# Autodesk Inventor assembly: forklift_1_0
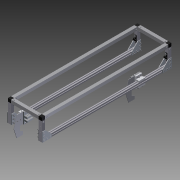
[picture p0: Inventor's stored thumbnail of the model, 180x180]
Saved by Autodesk Inventor 2011 (Build 150239000, 239)
## iProperties
Created: 2013-01-16
Part Number: forklift_1_0
Document SubType Name: Assembly
Designer: 917788
Author: 917788
## Documents named in this file (13)
- F:\Users\Christopher\Documents\GitHub\2013CAD\2013 robot\forklift\frame parts\forklift_1_0.iam
- F:\Users\Christopher\Documents\GitHub\2013CAD\2013 robot\forklift\frame parts\1tube_6.ipt
- F:\Users\Christopher\Documents\GitHub\2013CAD\2013 robot\forklift\frame parts\1tube_9.ipt
- F:\Users\Christopher\Documents\GitHub\2013CAD\2013 robot\forklift\frame parts\1tube_40.ipt
- F:\Users\Christopher\Documents\GitHub\2013CAD\2013 robot\forklift\frame parts\8020_40.ipt
- F:\Users\Christopher\Documents\GitHub\2013CAD\2013 robot\forklift\frame parts\8020_gussetplate.ipt
- F:\Users\Christopher\Documents\GitHub\2013CAD\COTS parts\Plastic_Tubing_Connectors\3-way corner.ipt
- F:\Users\Christopher\Documents\GitHub\2013CAD\COTS parts\Bearings\.5inch_side_bearing.ipt
- F:\Users\Christopher\Documents\GitHub\2013CAD\2013 robot\forklift\Misc parts\1.5_bolt_.25_20.ipt
- F:\Users\Christopher\Documents\GitHub\2013CAD\2013 robot\forklift\Misc parts\2_bolt_.25_20.ipt
- F:\Users\Christopher\Documents\GitHub\2013CAD\2013 robot\forklift\Misc parts\nut_.25_20.ipt
- F:\Users\Christopher\Documents\GitHub\2013CAD\2013 robot\forklift\frame parts\hook_right.iam
- F:\Users\Christopher\Documents\GitHub\2013CAD\2013 robot\forklift\frame parts\hook_left.iam
## Components (97 placed, 12 different names)
1. 1tube_9:1 — Mate:9, Mate:10, Flush:8, Mate:11, Mate:12, Flush:9, Insert:3, Insert:4, Insert:44, Insert:51
2. 1tube_40:1 — Mate:7, Flush:7, Mate:8, Mate:20, Mate:21, Flush:18, Insert:2, Insert:12, Insert:43
3. 8020_40:1 — Flush:22, Flush:24, Mate:41, Mate:42, Flush:28, Mate:49, Flush:38, Flush:39, Mate:57, Mate:58
4. 8020_gussetplate:1 — Mate:50, Flush:40, Flush:41, Insert:45, Insert:46, Insert:47, Insert:48, Insert:49
5. 1tube_40:2 — Mate:13, Mate:14, Flush:10, Mate:22, Mate:23, Mate:24, Insert:6, Insert:8, Insert:52, Insert:58
6. 1tube_9:2 — Mate:25, Mate:26, Mate:27, Insert:9, Insert:10, Insert:67, Insert:71
7. 1tube_6:2 — Mate:1, Flush:4, Flush:5, Mate:46, Flush:36, Mate:48, Flush:37, Insert:1, Insert:42
8. 8020_40:2 — Mate:1, Flush:3, Flush:6, Flush:20, Mate:39, Flush:34, Mate:47, Flush:35, Flush:37, Mate:59, Mate:60
9. 8020_gussetplate:2 — Flush:24, Mate:43, Flush:31, Flush:32, Insert:53, Insert:54, Insert:55, Insert:56, Insert:57
10. 8020_gussetplate:3 — Mate:55, Flush:42, Flush:43, Insert:27, Insert:28, Insert:29, Insert:30, Insert:31
11. 8020_gussetplate:4 — Flush:5, Flush:6, Mate:46, Flush:36, Insert:37, Insert:38, Insert:39, Insert:40, Insert:41
12. 8020_gussetplate:5 — Flush:3, Flush:4, Mate:48, Insert:17, Insert:18, Insert:19, Insert:20, Insert:21
13. 8020_gussetplate:7 — Flush:22, Flush:29, Flush:30, Insert:32, Insert:33, Insert:34, Insert:35, Insert:36
14. 8020_gussetplate:8 — Mate:31, Flush:19, Flush:20, Insert:22, Insert:23, Insert:24, Insert:25, Insert:26
15. 8020_gussetplate:9 — Mate:37, Flush:25, Flush:26, Insert:60, Insert:61, Insert:62, Insert:63, Insert:64
16. 3-way corner:1 — Mate:11, Mate:12, Flush:9, Mate:13, Mate:14, Flush:10, Mate:52, Mate:53, Mate:54
17. 3-way corner:2 — Mate:7, Flush:7, Mate:8, Mate:9, Mate:10, Flush:8
18. 3-way corner:3 — Mate:20, Mate:21, Flush:18, Mate:25, Mate:28, Mate:29, Mate:30
19. 3-way corner:4 — Mate:22, Mate:23, Mate:24, Mate:26, Mate:27, Mate:44, Mate:51
20. 1tube_6:4 — Mate:28, Mate:29, Mate:30, Mate:31, Flush:19, Mate:37, Flush:25, Flush:26, Mate:38, Flush:27, Flush:34, Mate:47, Flush:35, Insert:11, Insert:65, Insert:66, Insert:68
21. .5inch_side_bearing:1 — Mate:41, Flush:33, Mate:45, Insert:15, Insert:16
22. .5inch_side_bearing:2 — Mate:38, Flush:27, Mate:39, Insert:13, Insert:14
23. 1tube_6:5 — Mate:42, Mate:43, Flush:28, Flush:29, Flush:30, Flush:31, Flush:32, Flush:33, Mate:44, Mate:45, Mate:51, Insert:7, Insert:59, Insert:69, Insert:70
24. 1tube_6:6 — Mate:49, Flush:38, Flush:39, Mate:50, Mate:52, Mate:53, Mate:54, Flush:40, Flush:41, Mate:55, Flush:42, Flush:43, Insert:5, Insert:50
25. 1.5_bolt_.25_20:1 — Insert:2
26. 2_bolt_.25_20:1 — Insert:17
27. 1.5_bolt_.25_20:2 — Insert:1
28. 1.5_bolt_.25_20:3 — Insert:4
29. 1.5_bolt_.25_20:4 — Insert:3
30. 1.5_bolt_.25_20:5 — Insert:6
31. 1.5_bolt_.25_20:6 — Insert:11
32. 1.5_bolt_.25_20:7 — Insert:8
33. 1.5_bolt_.25_20:8 — Insert:9
34. 1.5_bolt_.25_20:9 — Insert:7
35. 1.5_bolt_.25_20:10 — Insert:10
36. 1.5_bolt_.25_20:11 — Insert:15
37. 1.5_bolt_.25_20:12 — Insert:16
38. 1.5_bolt_.25_20:13 — Insert:12
39. 1.5_bolt_.25_20:14 — Insert:5
40. 1.5_bolt_.25_20:15 — Insert:14
41. 1.5_bolt_.25_20:16 — Insert:13
42. 2_bolt_.25_20:2 — Insert:19
43. 2_bolt_.25_20:3 — Insert:18
44. 2_bolt_.25_20:4 — Insert:20
45. 2_bolt_.25_20:5 — Insert:27
46. 2_bolt_.25_20:6 — Insert:28
47. 2_bolt_.25_20:7 — Insert:21
48. 2_bolt_.25_20:8 — Insert:22
49. 2_bolt_.25_20:9 — Insert:23
50. 2_bolt_.25_20:10 — Insert:26
51. 2_bolt_.25_20:11 — Insert:24
52. 2_bolt_.25_20:12 — Insert:25
53. 2_bolt_.25_20:13 — Insert:35
54. 2_bolt_.25_20:14 — Insert:36
55. 2_bolt_.25_20:15 — Insert:34
56. 2_bolt_.25_20:16 — Insert:33
57. 2_bolt_.25_20:17 — Insert:32
58. 2_bolt_.25_20:18 — Insert:29
59. 2_bolt_.25_20:19 — Insert:30
60. 2_bolt_.25_20:20 — Insert:31
61. nut_.25_20:1 — Insert:37
62. nut_.25_20:2 — Insert:49
63. nut_.25_20:3 — Insert:46
64. nut_.25_20:4 — Insert:44
65. nut_.25_20:5 — Insert:45
66. nut_.25_20:6 — Insert:50
67. nut_.25_20:7 — Insert:43
68. nut_.25_20:8 — Insert:40
69. nut_.25_20:9 — Insert:52
70. nut_.25_20:10 — Insert:51
71. nut_.25_20:11 — Insert:53
72. nut_.25_20:12 — Insert:38
73. nut_.25_20:13 — Insert:39
74. nut_.25_20:14 — Insert:48
75. nut_.25_20:15 — Insert:47
76. nut_.25_20:16 — Insert:41
77. nut_.25_20:17 — Insert:42
78. nut_.25_20:18 — Insert:63
79. nut_.25_20:19 — Insert:54
80. nut_.25_20:20 — Insert:61
81. nut_.25_20:21 — Insert:62
82. nut_.25_20:22 — Insert:57
83. nut_.25_20:23 — Insert:60
84. nut_.25_20:24 — Insert:65
85. nut_.25_20:25 — Insert:66
86. nut_.25_20:26 — Insert:59
87. nut_.25_20:27 — Insert:56
88. nut_.25_20:28 — Insert:64
89. nut_.25_20:29 — Insert:69
90. nut_.25_20:30 — Insert:67
91. nut_.25_20:31 — Insert:55
92. nut_.25_20:32 — Insert:70
93. nut_.25_20:33 — Insert:58
94. nut_.25_20:34 — Insert:71
95. nut_.25_20:35 — Insert:68
96. hook_right:1 [sub-assembly] — Mate:57, Mate:58
97. hook_left:1 [sub-assembly] — Mate:59, Mate:60
## Relationships (146: Insert 71, Mate 43, Flush 32)
- Mate:1: 1tube_6:2 ↔ 8020_40:2
- Flush:3: 8020_40:2 ↔ 8020_gussetplate:5
- Flush:4: 1tube_6:2 ↔ 8020_gussetplate:5
- Flush:5: 1tube_6:2 ↔ 8020_gussetplate:4
- Flush:6: 8020_40:2 ↔ 8020_gussetplate:4
- Mate:7: 1tube_40:1 ↔ 3-way corner:2
- Flush:7: 1tube_40:1 ↔ 3-way corner:2
- Mate:8: 1tube_40:1 ↔ 3-way corner:2
- Mate:9: 1tube_9:1 ↔ 3-way corner:2
- Mate:10: 1tube_9:1 ↔ 3-way corner:2
- Flush:8: 1tube_9:1 ↔ 3-way corner:2
- Mate:11: 1tube_9:1 ↔ 3-way corner:1
- Mate:12: 1tube_9:1 ↔ 3-way corner:1
- Flush:9: 1tube_9:1 ↔ 3-way corner:1
- Mate:13: 1tube_40:2 ↔ 3-way corner:1
- Mate:14: 1tube_40:2 ↔ 3-way corner:1
- Flush:10: 1tube_40:2 ↔ 3-way corner:1
- Mate:20: 1tube_40:1 ↔ 3-way corner:3
- Mate:21: 1tube_40:1 ↔ 3-way corner:3
- Flush:18: 1tube_40:1 ↔ 3-way corner:3
- Mate:22: 1tube_40:2 ↔ 3-way corner:4
- Mate:23: 1tube_40:2 ↔ 3-way corner:4
- Mate:24: 1tube_40:2 ↔ 3-way corner:4
- Mate:25: 1tube_9:2 ↔ 3-way corner:3
- Mate:26: 1tube_9:2 ↔ 3-way corner:4
- Mate:27: 1tube_9:2 ↔ 3-way corner:4
- Mate:28: 3-way corner:3 ↔ 1tube_6:4
- Mate:29: 3-way corner:3 ↔ 1tube_6:4
- Mate:30: 3-way corner:3 ↔ 1tube_6:4
- Mate:31: 8020_gussetplate:8 ↔ 1tube_6:4
- Flush:19: 8020_gussetplate:8 ↔ 1tube_6:4
- Flush:20: 8020_40:2 ↔ 8020_gussetplate:8
- Flush:22: 8020_40:1 ↔ 8020_gussetplate:7
- Flush:24: 8020_40:1 ↔ 8020_gussetplate:2
- Mate:37: 8020_gussetplate:9 ↔ 1tube_6:4
- Flush:25: 8020_gussetplate:9 ↔ 1tube_6:4
- Flush:26: 8020_gussetplate:9 ↔ 1tube_6:4
- Mate:38: 1tube_6:4 ↔ .5inch_side_bearing:2
- Flush:27 (6.35 mm): 1tube_6:4 ↔ .5inch_side_bearing:2
- Mate:39 (38.1 mm): 8020_40:2 ↔ .5inch_side_bearing:2
- Mate:41 (38.1 mm): 8020_40:1 ↔ .5inch_side_bearing:1
- Mate:42: 8020_40:1 ↔ 1tube_6:5
- Mate:43: 8020_gussetplate:2 ↔ 1tube_6:5
- Flush:28: 8020_40:1 ↔ 1tube_6:5
- Flush:29: 8020_gussetplate:7 ↔ 1tube_6:5
- Flush:30: 8020_gussetplate:7 ↔ 1tube_6:5
- Flush:31: 8020_gussetplate:2 ↔ 1tube_6:5
- Flush:32: 8020_gussetplate:2 ↔ 1tube_6:5
- Flush:33 (6.35 mm): .5inch_side_bearing:1 ↔ 1tube_6:5
- Mate:44: 3-way corner:4 ↔ 1tube_6:5
- Mate:45: .5inch_side_bearing:1 ↔ 1tube_6:5
- Flush:34: 8020_40:2 ↔ 1tube_6:4
- Mate:46: 1tube_6:2 ↔ 8020_gussetplate:4
- Mate:47: 8020_40:2 ↔ 1tube_6:4
- Flush:35: 8020_40:2 ↔ 1tube_6:4
- Flush:36: 1tube_6:2 ↔ 8020_gussetplate:4
- Mate:48: 1tube_6:2 ↔ 8020_gussetplate:5
- Flush:37: 1tube_6:2 ↔ 8020_40:2
- Mate:49: 8020_40:1 ↔ 1tube_6:6
- Flush:38: 8020_40:1 ↔ 1tube_6:6
- Flush:39: 8020_40:1 ↔ 1tube_6:6
- Mate:50: 8020_gussetplate:1 ↔ 1tube_6:6
- Mate:51: 3-way corner:4 ↔ 1tube_6:5
- Mate:52: 3-way corner:1 ↔ 1tube_6:6
- Mate:53: 3-way corner:1 ↔ 1tube_6:6
- Mate:54: 3-way corner:1 ↔ 1tube_6:6
- Flush:40: 8020_gussetplate:1 ↔ 1tube_6:6
- Flush:41: 8020_gussetplate:1 ↔ 1tube_6:6
- Mate:55: 8020_gussetplate:3 ↔ 1tube_6:6
- Flush:42: 8020_gussetplate:3 ↔ 1tube_6:6
- Flush:43: 8020_gussetplate:3 ↔ 1tube_6:6
- Insert:1: 1tube_6:2 ↔ 1.5_bolt_.25_20:2
- Insert:2: 1tube_40:1 ↔ 1.5_bolt_.25_20:1
- Insert:3: 1tube_9:1 ↔ 1.5_bolt_.25_20:4
- Insert:4: 1tube_9:1 ↔ 1.5_bolt_.25_20:3
- Insert:5: 1tube_6:6 ↔ 1.5_bolt_.25_20:14
- Insert:6: 1tube_40:2 ↔ 1.5_bolt_.25_20:5
- Insert:7: 1tube_6:5 ↔ 1.5_bolt_.25_20:9
- Insert:8: 1tube_40:2 ↔ 1.5_bolt_.25_20:7
- Insert:9: 1tube_9:2 ↔ 1.5_bolt_.25_20:8
- Insert:10: 1tube_9:2 ↔ 1.5_bolt_.25_20:10
- Insert:11: 1tube_6:4 ↔ 1.5_bolt_.25_20:6
- Insert:12: 1tube_40:1 ↔ 1.5_bolt_.25_20:13
- Insert:13: .5inch_side_bearing:2 ↔ 1.5_bolt_.25_20:16
- Insert:14: .5inch_side_bearing:2 ↔ 1.5_bolt_.25_20:15
- Insert:15: .5inch_side_bearing:1 ↔ 1.5_bolt_.25_20:11
- Insert:16: .5inch_side_bearing:1 ↔ 1.5_bolt_.25_20:12
- Insert:17: 8020_gussetplate:5 ↔ 2_bolt_.25_20:1
- Insert:18: 8020_gussetplate:5 ↔ 2_bolt_.25_20:3
- Insert:19: 8020_gussetplate:5 ↔ 2_bolt_.25_20:2
- Insert:20: 8020_gussetplate:5 ↔ 2_bolt_.25_20:4
- Insert:21: 8020_gussetplate:5 ↔ 2_bolt_.25_20:7
- Insert:22: 8020_gussetplate:8 ↔ 2_bolt_.25_20:8
- Insert:23: 8020_gussetplate:8 ↔ 2_bolt_.25_20:9
- Insert:24: 8020_gussetplate:8 ↔ 2_bolt_.25_20:11
- Insert:25: 8020_gussetplate:8 ↔ 2_bolt_.25_20:12
- Insert:26: 8020_gussetplate:8 ↔ 2_bolt_.25_20:10
- Insert:27: 8020_gussetplate:3 ↔ 2_bolt_.25_20:5
- Insert:28: 8020_gussetplate:3 ↔ 2_bolt_.25_20:6
- Insert:29: 8020_gussetplate:3 ↔ 2_bolt_.25_20:18
- Insert:30: 8020_gussetplate:3 ↔ 2_bolt_.25_20:19
- Insert:31: 8020_gussetplate:3 ↔ 2_bolt_.25_20:20
- Insert:32: 8020_gussetplate:7 ↔ 2_bolt_.25_20:17
- Insert:33: 8020_gussetplate:7 ↔ 2_bolt_.25_20:16
- Insert:34: 8020_gussetplate:7 ↔ 2_bolt_.25_20:15
- Insert:35: 8020_gussetplate:7 ↔ 2_bolt_.25_20:13
- Insert:36: 8020_gussetplate:7 ↔ 2_bolt_.25_20:14
- Insert:37: 8020_gussetplate:4 ↔ nut_.25_20:1
- Insert:38: 8020_gussetplate:4 ↔ nut_.25_20:12
- Insert:39: 8020_gussetplate:4 ↔ nut_.25_20:13
- Insert:40: 8020_gussetplate:4 ↔ nut_.25_20:8
- Insert:41: 8020_gussetplate:4 ↔ nut_.25_20:16
- Insert:42: 1tube_6:2 ↔ nut_.25_20:17
- Insert:43: 1tube_40:1 ↔ nut_.25_20:7
- Insert:44: 1tube_9:1 ↔ nut_.25_20:4
- Insert:45: 8020_gussetplate:1 ↔ nut_.25_20:5
- Insert:46: 8020_gussetplate:1 ↔ nut_.25_20:3
- Insert:47: 8020_gussetplate:1 ↔ nut_.25_20:15
- Insert:48: 8020_gussetplate:1 ↔ nut_.25_20:14
- Insert:49: 8020_gussetplate:1 ↔ nut_.25_20:2
- Insert:50: 1tube_6:6 ↔ nut_.25_20:6
- Insert:51: 1tube_9:1 ↔ nut_.25_20:10
- Insert:52: 1tube_40:2 ↔ nut_.25_20:9
- Insert:53: 8020_gussetplate:2 ↔ nut_.25_20:11
- Insert:54: 8020_gussetplate:2 ↔ nut_.25_20:19
- Insert:55: 8020_gussetplate:2 ↔ nut_.25_20:31
- Insert:56: 8020_gussetplate:2 ↔ nut_.25_20:27
- Insert:57: 8020_gussetplate:2 ↔ nut_.25_20:22
- Insert:58: 1tube_40:2 ↔ nut_.25_20:33
- Insert:59: 1tube_6:5 ↔ nut_.25_20:26
- Insert:60: 8020_gussetplate:9 ↔ nut_.25_20:23
- Insert:61: 8020_gussetplate:9 ↔ nut_.25_20:20
- Insert:62: 8020_gussetplate:9 ↔ nut_.25_20:21
- Insert:63: 8020_gussetplate:9 ↔ nut_.25_20:18
- Insert:64: 8020_gussetplate:9 ↔ nut_.25_20:28
- Insert:65: 1tube_6:4 ↔ nut_.25_20:24
- Insert:66: 1tube_6:4 ↔ nut_.25_20:25
- Insert:67: 1tube_9:2 ↔ nut_.25_20:30
- Insert:68: 1tube_6:4 ↔ nut_.25_20:35
- Insert:69: 1tube_6:5 ↔ nut_.25_20:29
- Insert:70: 1tube_6:5 ↔ nut_.25_20:32
- Insert:71: 1tube_9:2 ↔ nut_.25_20:34
- Mate:57: 8020_40:1 ↔ hook_right:1
- Mate:58: 8020_40:1 ↔ hook_right:1
- Mate:59: 8020_40:2 ↔ hook_left:1
- Mate:60: 8020_40:2 ↔ hook_left:1
